# Autodesk Inventor assembly: motor
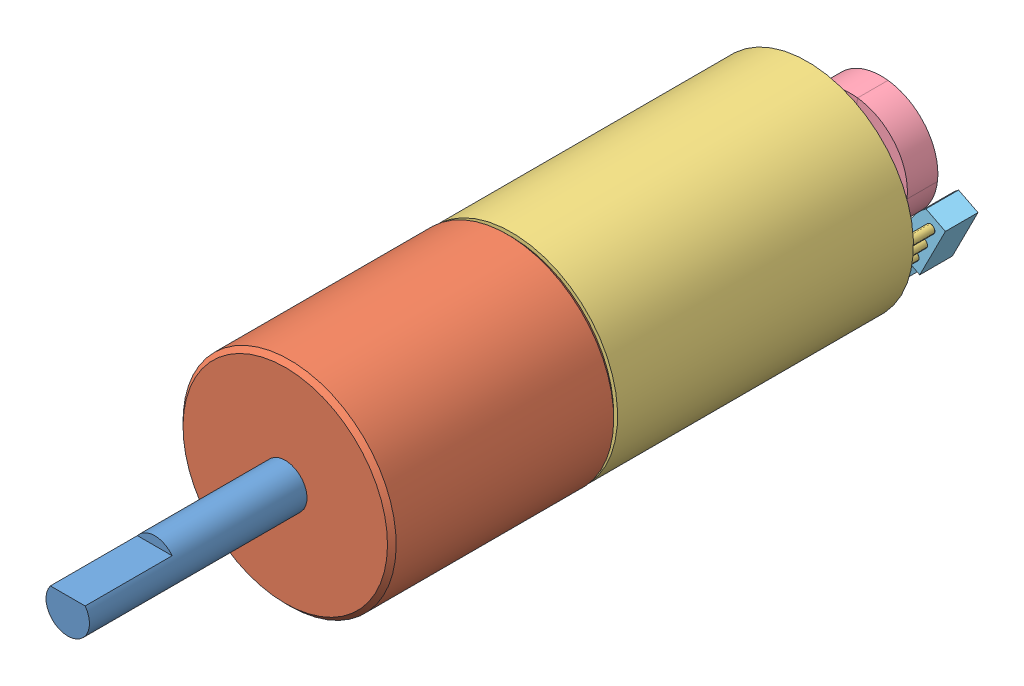
[picture p0: shaded view drawn from the part files that the assembly names]
Saved by Autodesk Inventor 2019.4 (Build 234330000, 330)
## iProperties
Created: 2020-06-20
Part Number: motor
Document SubType Name: Assembly
Designer: Jorge
Author: Jorge
## Documents named in this file (4)
- D:\TFG\dev\hardware\ROVER\motor.iam
- D:\TFG\dev\hardware\ROVER\shaft.ipt
- D:\TFG\dev\hardware\ROVER\gearbox.ipt
- D:\TFG\dev\hardware\ROVER\motor_core.iam
## Components (3 placed, 3 different names)
1. shaft:1 — Mate:1, Mate:2, Rotation:1
2. gearbox:1 — Mate:1, Mate:2, Mate:3, Mate:4
3. motor_core:1 [sub-assembly] — Mate:3, Mate:4, Rotation:1
## Relationships (5: Mate 4, RelateRotation 1)
- Mate:1: shaft:1 ↔ gearbox:1
- Mate:2: shaft:1 ↔ gearbox:1
- Mate:3: gearbox:1 ↔ motor_core:1
- Mate:4: gearbox:1 ↔ motor_core:1
- Rotation:1 [RelateRotation] (1 ul): shaft:1 ↔ motor_core:1
